# Autodesk Inventor assembly: gear-assembly
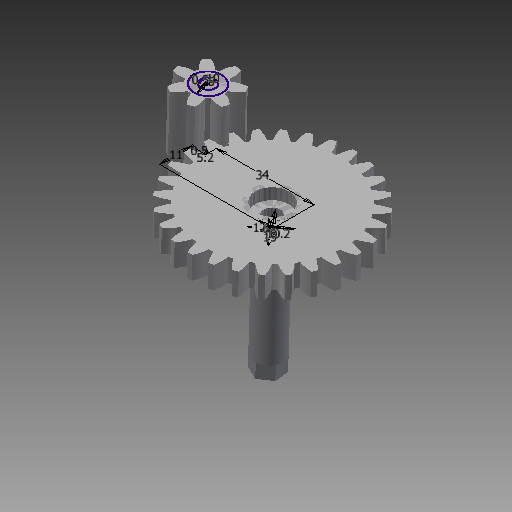
[picture p0: Inventor's stored thumbnail of the model, 512x512]
Saved by Autodesk Inventor 2017 (Build 210142000, 142)
## iProperties
Created: 2026-03-25
Part Number: gear-assembly
Document SubType Name: Assembly
Designer: a
Author: a
## Documents named in this file (5)
- C:\Users\a\Documents\the-claw-pnp\gear-assembly.iam
- C:\Users\a\Documents\the-claw-pnp\vacuum-gear-shaft.ipt
- C:\Users\a\Documents\the-claw-pnp\motor-gear-base.ipt
- C:\Users\a\Documents\the-claw-pnp\literally-just-a-sketch.ipt
- C:\Users\a\Documents\the-claw-pnp\gear-assembly\Design Accelerator\Spur Gears1.iam
## Components (4 placed, 4 different names)
1. vacuum-gear-shaft:1 — Mate:2, Flush:1, Mate:5, Flush:3
2. motor-gear-base:1 — Mate:3, Flush:1, Mate:4, Flush:2
3. literally-just-a-sketch:1 — Mate:2, Mate:3
4. Spur Gears:1 [sub-assembly] — Mate:4, Flush:2, Mate:5, Flush:3
## Relationships (7: Mate 4, Flush 3)
- Mate:2: vacuum-gear-shaft:1 ↔ literally-just-a-sketch:1
- Mate:3: motor-gear-base:1 ↔ literally-just-a-sketch:1
- Flush:1: vacuum-gear-shaft:1 ↔ motor-gear-base:1
- Mate:4: motor-gear-base:1 ↔ Spur Gears:1
- Flush:2: motor-gear-base:1 ↔ Spur Gears:1
- Mate:5: vacuum-gear-shaft:1 ↔ Spur Gears:1
- Flush:3: vacuum-gear-shaft:1 ↔ Spur Gears:1
